# Autodesk Inventor assembly: Idler Wheel
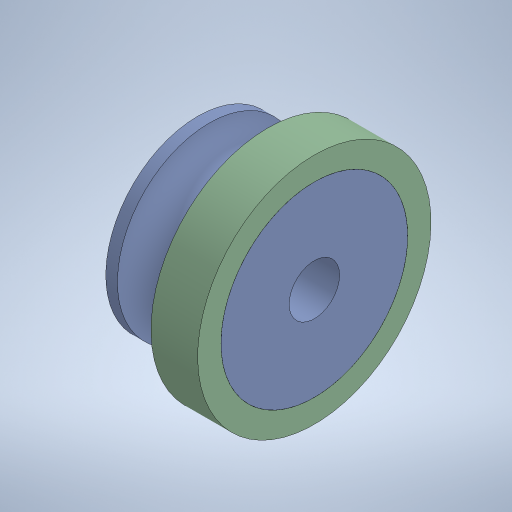
[picture p0: Inventor's stored thumbnail of the model, 512x512]
Saved by Autodesk Inventor 2023.2 (Build 272271000, 271)
## iProperties
Created: 2023-11-16
Part Number: Idler Wheel
Document SubType Name: Assembly
Designer: Nathan Cai
Author: Nathan Cai
## Documents named in this file (3)
- E:\Documents\Inventor\Chort V2.0\Idler Wheel.iam
- E:\Documents\Inventor\Chort V2.0\Idler - Puley.ipt
- E:\Documents\Inventor\Chort V2.0\Idler - Tire.ipt
## Components (2 placed, 2 different names)
1. Idler - Puley:1 — Mate:1, Flush:1
2. Idler - Tire:1 — Mate:1, Flush:1
## Relationships (2: Mate 1, Flush 1)
- Mate:1: Idler - Puley:1 ↔ Idler - Tire:1
- Flush:1: Idler - Puley:1 ↔ Idler - Tire:1
